# Autodesk Inventor assembly: booth
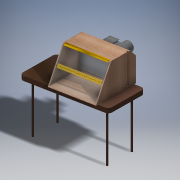
[picture p0: Inventor's stored thumbnail of the model, 180x180]
Saved by Autodesk Inventor 2017 (Build 210142000, 142)
## iProperties
Created: 2019-04-11
Part Number: booth
Document SubType Name: Assembly
Designer: Brian
Author: Brian
## Documents named in this file (25)
- B:\Miniatures\spray booth\booth.iam
- B:\Miniatures\spray booth\Frame - Horizontal (Bottom Front).ipt
- B:\Miniatures\spray booth\Frame - Horizontal (Bottom Rear).ipt
- B:\Miniatures\spray booth\Frame - Horizontal (Top Front).ipt
- B:\Miniatures\spray booth\Frame - Horizontal (Top Rear).ipt
- B:\Miniatures\spray booth\Back Side.ipt
- B:\Miniatures\spray booth\Cap Side.ipt
- B:\Miniatures\spray booth\Frame - Vertical (Clones).ipt
- B:\Miniatures\spray booth\Frame - Vertical (Left Front).ipt
- B:\Miniatures\spray booth\Two By Four - Rectangle.ipt
- B:\Miniatures\spray booth\Two By Four - Triangle.ipt
- B:\Miniatures\spray booth\Top Side.ipt
- B:\Miniatures\spray booth\Left Side.ipt
- B:\Miniatures\spray booth\Bottom Base.ipt
- B:\Miniatures\spray booth\Right Side - Rear.ipt
- B:\Miniatures\spray booth\Right Side - Forward.ipt
- B:\Miniatures\spray booth\Filter.ipt
- B:\Miniatures\spray booth\Acrylic Panel - Top.ipt
- B:\Miniatures\spray booth\Acrylic Panel - Bottom.ipt
- B:\Miniatures\spray booth\PianoHingePlate.ipt
- B:\Miniatures\spray booth\PianoHingePin.ipt
- B:\Miniatures\spray booth\dayton1TDT2 $167.ipt
- B:\Miniatures\spray booth\table.ipt
- B:\Miniatures\spray booth\textures\Wrinkled Paper.jpg
- B:\Miniatures\spray booth\textures\images.png
## Components (26 placed, 22 different names)
1. Frame - Horizontal (Bottom Front):1 — Slider:1
2. Frame - Horizontal (Bottom Rear):1
3. Frame - Horizontal (Top Front):1
4. Frame - Horizontal (Top Rear):1
5. Back Side:1 — Mate:14
6. Cap Side:1
7. Frame - Vertical (Clones):1
8. Frame - Vertical (Left Front):1
9. Two By Four - Rectangle:1
10. Two By Four - Triangle:1
11. Top Side:1 — Mate:2, Flush:4
12. Left Side:1
13. Bottom Base:1 — Slider:2
14. Right Side - Rear:1
15. Right Side - Forward:1 — Mate:4, Mate:9
16. Filter:1 — Slider:1
17. Acrylic Panel - Top:1 — Flush:1, Mate:7, Mate:8, Mate:10, Flush:2, Mate:11
18. Acrylic Panel - Bottom:1 — Mate:12, Flush:3, Mate:13
19. PianoHingePlate:1 — Flush:1, Mate:7, Mate:8, Rotational:1, Insert:1
20. PianoHingePlate:2 — Mate:2, Mate:4, Rotational:1, Mate:9
21. PianoHingePin:1 — Insert:1
22. PianoHingePlate:3 — Mate:10, Flush:2, Mate:11, Rotational:2, Insert:2
23. PianoHingePlate:4 — Rotational:2, Mate:12, Flush:3, Mate:13
24. PianoHingePin:2 — Insert:2
25. dayton1TDT2 $167:2 — Mate:14, Flush:4
26. table:1 — Slider:2
## Relationships (20: Mate 10, Flush 4, TranslationJoint 2, RevoluteJoint 2, Insert 2)
- Slider:1 [TranslationJoint]: Frame - Horizontal (Bottom Front):1 ↔ Filter:1
- Mate:2: Top Side:1 ↔ PianoHingePlate:2
- Mate:4 (25.4 mm): Right Side - Forward:1 ↔ PianoHingePlate:2
- Flush:1 (25.4 mm): Acrylic Panel - Top:1 ↔ PianoHingePlate:1
- Mate:7: Acrylic Panel - Top:1 ↔ PianoHingePlate:1
- Mate:8: Acrylic Panel - Top:1 ↔ PianoHingePlate:1
- Rotational:1 [RevoluteJoint]: PianoHingePlate:1 ↔ PianoHingePlate:2
- Mate:9 (6.35 mm): Right Side - Forward:1 ↔ PianoHingePlate:2
- Insert:1: PianoHingePlate:1 ↔ PianoHingePin:1
- Mate:10: Acrylic Panel - Top:1 ↔ PianoHingePlate:3
- Flush:2 (25.4 mm): Acrylic Panel - Top:1 ↔ PianoHingePlate:3
- Mate:11: Acrylic Panel - Top:1 ↔ PianoHingePlate:3
- Rotational:2 [RevoluteJoint]: PianoHingePlate:3 ↔ PianoHingePlate:4
- Mate:12: Acrylic Panel - Bottom:1 ↔ PianoHingePlate:4
- Flush:3 (25.4 mm): Acrylic Panel - Bottom:1 ↔ PianoHingePlate:4
- Mate:13: Acrylic Panel - Bottom:1 ↔ PianoHingePlate:4
- Insert:2: PianoHingePlate:3 ↔ PianoHingePin:2
- Mate:14: Back Side:1 ↔ dayton1TDT2 $167:2
- Flush:4 (88.9 mm): Top Side:1 ↔ dayton1TDT2 $167:2
- Slider:2 [TranslationJoint]: Bottom Base:1 ↔ table:1
